# Autodesk Inventor assembly: MG-Mainboard
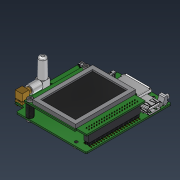
[picture p0: Inventor's stored thumbnail of the model, 180x180]
Saved by Autodesk Inventor 2022.1 (Build 261234020, 234B)
## iProperties
Part Number: MG-Mainboard
Material: Generisch
Document SubType Name: Assembly
Designer: rYan
Mass: 55.9255 g
Surface Area: 380.217 cm^2
Volume: 31.4122 cm^3
Density: 1.78037 g/cm^3
Author: rYan
## Documents named in this file (16)
- D:\TIGERsGIT\Hardware\mechanik\2020\Inventor\Robot\Electronics\MG-Mainboard.iam
- D:\TIGERsGIT\Hardware\mechanik\2020\Inventor\Robot\Electronics\Mainboard.ipt
- D:\TIGERsGIT\Hardware\mechanik\2020\Inventor\Purchased Parts\MG-LT24.iam
- D:\TIGERsGIT\Hardware\mechanik\2020\Inventor\Purchased Parts\SDCard TE.ipt
- D:\TIGERsGIT\Hardware\mechanik\2020\Inventor\Purchased Parts\USB A Female.ipt
- D:\TIGERsGIT\Hardware\mechanik\2020\Inventor\Purchased Parts\TSM-120-01-T-DV-P\TSM-120-01-T-DV-P.iam
- D:\TIGERsGIT\Hardware\mechanik\2020\Inventor\Purchased Parts\Abstandsbolzen Typ A M3-12mm.ipt
- D:\TIGERsGIT\Hardware\mechanik\2019\Inventor\Kaufteile\Abstandsbolzen Typ A.ipt
- D:\TIGERsGIT\Hardware\mechanik\2020\Inventor\Inhaltscenter\de-DE\DIN 7984\DIN 7984 - M3 x 5.ipt
- D:\TIGERsGIT\Hardware\mechanik\2020\Inventor\Purchased Parts\TE FFC Con 8pin 1mm vertical.ipt
- D:\TIGERsGIT\Hardware\mechanik\2020\Inventor\Purchased Parts\TE FFC Con 40pin 0.5mm bottom.ipt
- D:\TIGERsGIT\Hardware\mechanik\2020\Inventor\Purchased Parts\Antenne-Klein.ipt
- D:\TIGERsGIT\Hardware\mechanik\2020\Inventor\Purchased Parts\KT11P4.ipt
- D:\TIGERsGIT\Hardware\mechanik\2020\Inventor\Purchased Parts\SMA-F-RA.ipt
- D:\TIGERsGIT\Hardware\mechanik\2020\Inventor\Purchased Parts\TE FFC Con 10pin 1mm bottom.ipt
- D:\TIGERsGIT\Hardware\mechanik\2020\Inventor\Purchased Parts\Spacer M2 3mm.ipt
## Components (20 placed, 14 different names)
1. Mainboard:1 — Fluchtend:1, Fluchtend:2, Fluchtend:3, Passend:2, Fluchtend:8, Passend:6, Fluchtend:10, Passend:8, Einfügen:1, Einfügen:2, Einfügen:3, Einfügen:7, Passend:12, Fluchtend:14, Passend:15, Fluchtend:16, Passend:19, Fluchtend:17, Passend:20, Passend:21, Fluchtend:18, Passend:22, Passend:23, Passend:24, Passend:25, Passend:26, Einfügen:16, Einfügen:17, Einfügen:18
2. MG-LT24:1 [sub-assembly] — Passend:9, Fluchtend:12, Fluchtend:13, Einfügen:5, Einfügen:6, Passend:10, Passend:11
3. SDCard TE:1 — Passend:2, Fluchtend:8, Passend:21
4. USB A Female:1 — Passend:6, Fluchtend:10, Fluchtend:18
5. TSM-120-01-T-DV-P:1 [sub-assembly] — Passend:8, Passend:9, Fluchtend:12, Fluchtend:13
6. Abstandsbolzen Typ A M3-12mm:1 — Einfügen:1, Passend:10
7. Abstandsbolzen Typ A M3-12mm:2 — Einfügen:2, Passend:11
8. DIN 7984 M3 x 5:1 — Einfügen:3
9. DIN 7984 M3 x 5:2 — Einfügen:7
10. DIN 7984 M3 x 5:3 — Einfügen:5
11. DIN 7984 M3 x 5:4 — Einfügen:6
12. TE FFC Con 8pin 1mm vertical:1 — Passend:12, Fluchtend:14, Fluchtend:15
13. TE FFC Con 40pin 0.5mm bottom:1 — Passend:15, Passend:16, Fluchtend:16
14. KT11P4:1 — Passend:19, Fluchtend:17
15. SMA-F-RA:1 — Einfügen:15, Passend:20, Winkel:1, Passend:22, Passend:23
16. Antenne-Klein:2 — Einfügen:15, Winkel:1
17. TE FFC Con 10pin 1mm bottom:1 — Passend:24, Passend:25, Passend:26
18. Spacer M2 3mm:1 — Einfügen:18
19. Spacer M2 3mm:2 — Einfügen:16
20. Spacer M2 3mm:3 — Einfügen:17
## Relationships (40: Mate 17, Flush 12, Insert 10, Angle 1)
- Fluchtend:1 [Flush]: Mainboard:1
- Fluchtend:2 [Flush]: Mainboard:1
- Fluchtend:3 [Flush]: Mainboard:1
- Passend:2 [Mate]: Mainboard:1 ↔ SDCard TE:1
- Fluchtend:8 [Flush]: Mainboard:1 ↔ SDCard TE:1
- Passend:6 [Mate]: Mainboard:1 ↔ USB A Female:1
- Fluchtend:10 [Flush]: Mainboard:1 ↔ USB A Female:1
- Passend:8 [Mate]: Mainboard:1 ↔ TSM-120-01-T-DV-P:1
- Passend:9 [Mate]: MG-LT24:1 ↔ TSM-120-01-T-DV-P:1
- Fluchtend:12 [Flush] (0.05 mm): MG-LT24:1 ↔ TSM-120-01-T-DV-P:1
- Fluchtend:13 [Flush] (-0.25 mm): MG-LT24:1 ↔ TSM-120-01-T-DV-P:1
- Einfügen:1 [Insert]: Mainboard:1 ↔ Abstandsbolzen Typ A M3-12mm:1
- Einfügen:2 [Insert]: Mainboard:1 ↔ Abstandsbolzen Typ A M3-12mm:2
- Einfügen:3 [Insert]: Mainboard:1 ↔ DIN 7984 M3 x 5:1
- Einfügen:5 [Insert]: MG-LT24:1 ↔ DIN 7984 M3 x 5:3
- Einfügen:6 [Insert]: MG-LT24:1 ↔ DIN 7984 M3 x 5:4
- Passend:10 [Mate]: MG-LT24:1 ↔ Abstandsbolzen Typ A M3-12mm:1
- Passend:11 [Mate]: MG-LT24:1 ↔ Abstandsbolzen Typ A M3-12mm:2
- Einfügen:7 [Insert]: Mainboard:1 ↔ DIN 7984 M3 x 5:2
- Passend:12 [Mate]: Mainboard:1 ↔ TE FFC Con 8pin 1mm vertical:1
- Fluchtend:14 [Flush] (28 mm): Mainboard:1 ↔ TE FFC Con 8pin 1mm vertical:1
- Fluchtend:15 [Flush] (36.5 mm): TE FFC Con 8pin 1mm vertical:1
- Passend:15 [Mate]: Mainboard:1 ↔ TE FFC Con 40pin 0.5mm bottom:1
- Passend:16 [Mate] (3 mm): TE FFC Con 40pin 0.5mm bottom:1
- Fluchtend:16 [Flush]: Mainboard:1 ↔ TE FFC Con 40pin 0.5mm bottom:1
- Passend:19 [Mate]: Mainboard:1 ↔ KT11P4:1
- Fluchtend:17 [Flush]: Mainboard:1 ↔ KT11P4:1
- Einfügen:15 [Insert] (-5 mm): SMA-F-RA:1 ↔ Antenne-Klein:2
- Passend:20 [Mate]: Mainboard:1 ↔ SMA-F-RA:1
- Winkel:1 [Angle] (0 deg): SMA-F-RA:1 ↔ Antenne-Klein:2
- Passend:21 [Mate] (37 mm): Mainboard:1 ↔ SDCard TE:1
- Fluchtend:18 [Flush] (-33 mm): Mainboard:1 ↔ USB A Female:1
- Passend:22 [Mate] (-6 mm): Mainboard:1 ↔ SMA-F-RA:1
- Passend:23 [Mate] (-23 mm): Mainboard:1 ↔ SMA-F-RA:1
- Passend:24 [Mate]: Mainboard:1 ↔ TE FFC Con 10pin 1mm bottom:1
- Passend:25 [Mate] (31 mm): Mainboard:1 ↔ TE FFC Con 10pin 1mm bottom:1
- Passend:26 [Mate] (16 mm): Mainboard:1 ↔ TE FFC Con 10pin 1mm bottom:1
- Einfügen:16 [Insert]: Mainboard:1 ↔ Spacer M2 3mm:2
- Einfügen:17 [Insert]: Mainboard:1 ↔ Spacer M2 3mm:3
- Einfügen:18 [Insert]: Mainboard:1 ↔ Spacer M2 3mm:1
